# Autodesk Inventor assembly: Rbiceps+servos
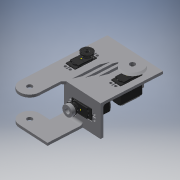
[picture p0: Inventor's stored thumbnail of the model, 180x180]
Saved by Autodesk Inventor 2018 (Build 220112000, 112)
## iProperties
Created: 2018-02-07
Part Number: Rbiceps+servos
Material: Générique
Document SubType Name: Assembly
Designer: Thomas
Author: Thomas
## Documents named in this file (5)
- D:\Users\Thomas\Desktop\Projet robot augmenté\robotConcept\Right biceps\Rbiceps+servos.iam
- D:\Users\Thomas\Desktop\Projet robot augmenté\robotConcept\Right biceps\Rbiceps.ipt
- D:\Users\Thomas\Desktop\Projet robot augmenté\robotConcept\MG996R SERVO\MG_996R.iam
- D:\Users\Thomas\Desktop\Projet robot augmenté\robotConcept\Wrist polley\Wrist polley.ipt
- D:\Users\Thomas\Desktop\Projet robot augmenté\robotConcept\Arm rotation\Arm rotation.ipt
## Components (7 placed, 4 different names)
1. Rbiceps:1 — Placage:1, Rotation:1, Rotation:2, Placage:2, Rotation:3, Rotation:4, Placage:3, Rotation:5, Placage:4, Rotation:6
2. MG_996R:1 [sub-assembly] — Placage:3, Rotation:5, Placage:5, Rotation:7
3. MG_996R:2 [sub-assembly] — Placage:2, Rotation:3, Rotation:4
4. MG_996R:3 [sub-assembly] — Placage:4, Rotation:6, Placage:6, Rotation:8
5. MG_996R:4 [sub-assembly] — Placage:1, Rotation:1, Rotation:2
6. Wrist polley:1 — Placage:5, Rotation:7
7. Arm rotation:1 — Placage:6, Rotation:8
## Relationships (14: RevoluteJoint 8, Mate 6)
- Placage:1 [Mate]: Rbiceps:1 ↔ MG_996R:4
- Rotation:1 [RevoluteJoint]: Rbiceps:1 ↔ MG_996R:4
- Rotation:2 [RevoluteJoint]: Rbiceps:1 ↔ MG_996R:4
- Placage:2 [Mate]: Rbiceps:1 ↔ MG_996R:2
- Rotation:3 [RevoluteJoint]: Rbiceps:1 ↔ MG_996R:2
- Rotation:4 [RevoluteJoint]: Rbiceps:1 ↔ MG_996R:2
- Placage:3 [Mate]: Rbiceps:1 ↔ MG_996R:1
- Rotation:5 [RevoluteJoint]: Rbiceps:1 ↔ MG_996R:1
- Placage:4 [Mate]: Rbiceps:1 ↔ MG_996R:3
- Rotation:6 [RevoluteJoint]: Rbiceps:1 ↔ MG_996R:3
- Placage:5 [Mate]: MG_996R:1 ↔ Wrist polley:1
- Rotation:7 [RevoluteJoint]: MG_996R:1 ↔ Wrist polley:1
- Placage:6 [Mate]: MG_996R:3 ↔ Arm rotation:1
- Rotation:8 [RevoluteJoint]: MG_996R:3 ↔ Arm rotation:1
